# Autodesk Inventor assembly: 6P 8T Sprocket, No Insert Right
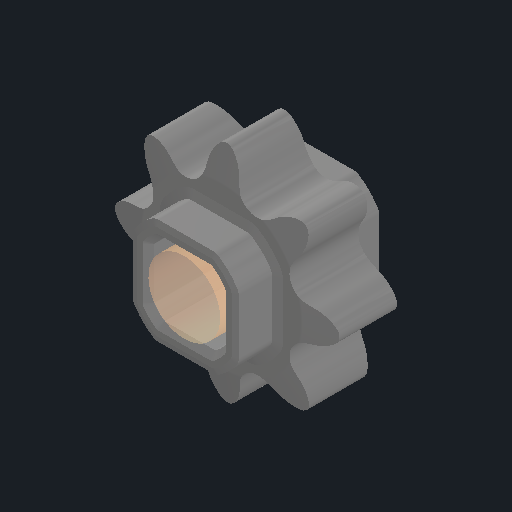
[picture p0: Inventor's stored thumbnail of the model, 512x512]
Saved by Autodesk Inventor 2025 (Build 290162000, 162)
## iProperties
Created: 2022-08-02
Part Number: 6P 8T Sprocket, No Insert Right
Document SubType Name: Assembly
Designer: Averey Ku
Author: ylu12
## Documents named in this file (2)
- D:\VEX\High Stakes\CAD\V2\Chassis\Drivebay Right\6P 8T Sprocket, No Insert Right.iam
- D:\VEX\High Stakes\CAD\V2\Chassis\Drivebay Right\6P 8T Sprocket Right.ipt
## Components (1 placed, 1 different names)
1. 6P 8T Sprocket Right:1 — Flush:3, Mate:6, Mate:5
## Relationships (3: Mate 2, Flush 1)
- Flush:3: 6P 8T Sprocket Right:1
- Mate:6: 6P 8T Sprocket Right:1
- Mate:5: 6P 8T Sprocket Right:1
